# Autodesk Inventor assembly: V-Belt transmission
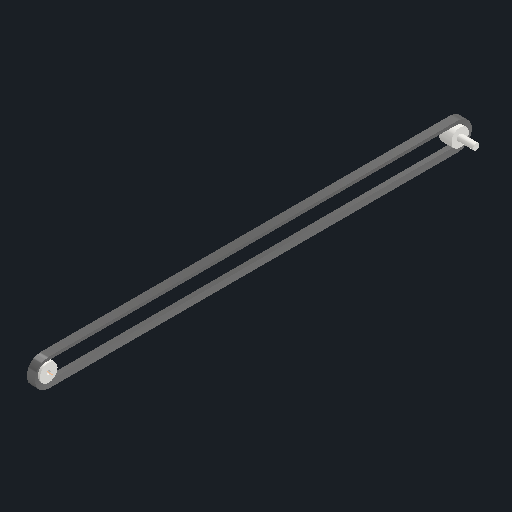
[picture p0: Inventor's stored thumbnail of the model, 512x512]
Saved by Autodesk Inventor 2024.2 (Build 282272000, 272)
## iProperties
ClientObjectVersion: 1
Created: 2024-03-22
Part Number: V-Belt transmission
Document SubType Name: Assembly
Designer: LightStore
Author: LightStore
## Documents named in this file (4)
- C:\Users\seifs\Downloads\Right Side Assembly\V-Belt transmission4.iam
- C:\Users\seifs\Downloads\Right Side Assembly\V-Belt4.ipt
- C:\Users\seifs\Downloads\Right Side Assembly\Flat Pulley11.ipt
- C:\Users\seifs\Downloads\Right Side Assembly\Flat Pulley21.ipt
## Components (3 placed, 3 different names)
1. V-Belt:1 — Flush:1, Mate:1, Flush:2, Mate:2
2. Flat Pulley1:1 — Flush:1, Mate:1, Rotation:1
3. Flat Pulley2:1 — Flush:2, Mate:2, Rotation:1
## Relationships (5: Flush 2, Mate 2, RelateRotation 1)
- Flush:1: V-Belt:1 ↔ Flat Pulley1:1
- Mate:1: V-Belt:1 ↔ Flat Pulley1:1
- Flush:2: V-Belt:1 ↔ Flat Pulley2:1
- Mate:2: V-Belt:1 ↔ Flat Pulley2:1
- Rotation:1 [RelateRotation] (1 ul): Flat Pulley1:1 ↔ Flat Pulley2:1
